# Autodesk Inventor assembly: B_Legs0
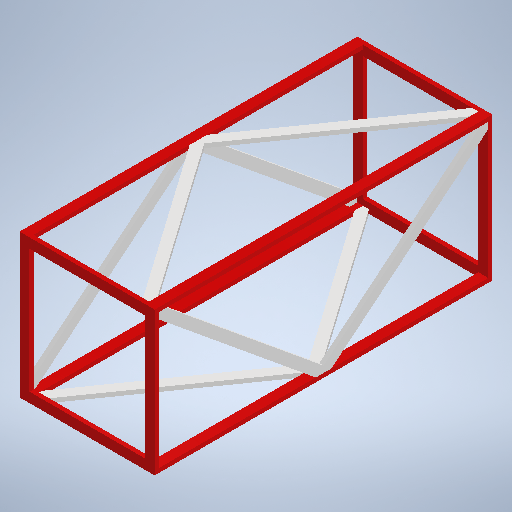
[picture p0: Inventor's stored thumbnail of the model, 512x512]
Saved by Autodesk Inventor 2025.1 (Build 291241020, 241B)
## iProperties
Created: 2024-09-19
Part Number: B_Legs0
Document SubType Name: Assembly
Designer: User
Author: User
## Documents named in this file (6)
- C:\Users\User\Documents\Tburn24\F_Legs1\B_Legs0.iam
- C:\Users\User\Documents\Tburn24\F_Legs1\8'x2x4.ipt
- C:\Users\User\Documents\Tburn24\F_Legs1\3'5x2x4.ipt
- C:\Users\User\Documents\Tburn24\F_Legs1\4x2x4.ipt
- C:\Users\User\Documents\Tburn24\F_Legs1\side1.ipt
- C:\Users\User\Documents\Tburn24\F_Legs1\side2.ipt
## Components (16 placed, 5 different names)
1. 8'x2x4:1 — Flush:1, Flush:2, Flush:3, Flush:8, Mate:3, Flush:10, Flush:12, Flush:13, Flush:14, Flush:22
2. 8'x2x4:2 — Mate:1, Flush:1, Flush:2, Flush:3, Mate:5, Flush:9, Flush:11, Flush:15, Flush:16, Flush:27, Mate:19, Flush:31, Mate:21, Flush:32
3. 4x2x4:1 — Flush:8, Flush:13, Flush:14, Mate:7, Flush:17, Flush:20, Mate:14, Mate:15, Flush:21, Mate:16, Flush:23, Flush:29
4. 4x2x4:2 — Mate:5, Flush:15, Flush:16, Mate:6, Flush:18, Flush:19, Mate:22
5. 4x2x4:3 — Flush:9, Flush:11, Flush:25, Flush:26
6. 4x2x4:4 — Mate:3, Flush:10, Flush:12, Mate:17, Mate:18
7. 8'x2x4:3 — Mate:7, Flush:17, Flush:20, Mate:14, Flush:24, Flush:30
8. 8'x2x4:4 — Mate:6, Flush:18, Flush:19, Flush:28
9. 3'5x2x4:1 — Mate:15, Flush:21, Flush:22
10. 3'5x2x4:2 — Mate:16, Flush:23, Flush:24
11. 3'5x2x4:3 — Mate:18, Flush:25, Flush:28
12. 3'5x2x4:4 — Mate:17, Flush:26, Flush:27, Mate:20
13. side1:1 — Flush:29
14. side2:1 — Flush:30
15. side2:2 — Mate:19, Mate:20, Flush:31
16. side1:2 — Mate:21, Mate:22, Flush:32
## Relationships (42: Flush 28, Mate 14)
- Mate:1: 8'x2x4:2
- Flush:1: 8'x2x4:1 ↔ 8'x2x4:2
- Flush:2 (1130.3 mm): 8'x2x4:1 ↔ 8'x2x4:2
- Flush:3: 8'x2x4:1 ↔ 8'x2x4:2
- Flush:8: 8'x2x4:1 ↔ 4x2x4:1
- Mate:3: 8'x2x4:1 ↔ 4x2x4:4
- Mate:5: 8'x2x4:2 ↔ 4x2x4:2
- Flush:9: 8'x2x4:2 ↔ 4x2x4:3
- Flush:10: 8'x2x4:1 ↔ 4x2x4:4
- Flush:11: 8'x2x4:2 ↔ 4x2x4:3
- Flush:12: 8'x2x4:1 ↔ 4x2x4:4
- Flush:13: 8'x2x4:1 ↔ 4x2x4:1
- Flush:14: 8'x2x4:1 ↔ 4x2x4:1
- Flush:15: 8'x2x4:2 ↔ 4x2x4:2
- Flush:16: 8'x2x4:2 ↔ 4x2x4:2
- Mate:6: 4x2x4:2 ↔ 8'x2x4:4
- Mate:7: 4x2x4:1 ↔ 8'x2x4:3
- Flush:17: 4x2x4:1 ↔ 8'x2x4:3
- Flush:18: 4x2x4:2 ↔ 8'x2x4:4
- Flush:19: 4x2x4:2 ↔ 8'x2x4:4
- Flush:20: 4x2x4:1 ↔ 8'x2x4:3
- Mate:14: 4x2x4:1 ↔ 8'x2x4:3
- Mate:15: 4x2x4:1 ↔ 3'5x2x4:1
- Flush:21: 4x2x4:1 ↔ 3'5x2x4:1
- Flush:22: 8'x2x4:1 ↔ 3'5x2x4:1
- Mate:16: 4x2x4:1 ↔ 3'5x2x4:2
- Flush:23: 4x2x4:1 ↔ 3'5x2x4:2
- Flush:24: 8'x2x4:3 ↔ 3'5x2x4:2
- Mate:17: 4x2x4:4 ↔ 3'5x2x4:4
- Mate:18: 4x2x4:4 ↔ 3'5x2x4:3
- Flush:25: 4x2x4:3 ↔ 3'5x2x4:3
- Flush:26: 4x2x4:3 ↔ 3'5x2x4:4
- Flush:27: 8'x2x4:2 ↔ 3'5x2x4:4
- Flush:28: 8'x2x4:4 ↔ 3'5x2x4:3
- Flush:29: 4x2x4:1 ↔ side1:1
- Flush:30: 8'x2x4:3 ↔ side2:1
- Mate:19: 8'x2x4:2 ↔ side2:2
- Mate:20: 3'5x2x4:4 ↔ side2:2
- Flush:31: 8'x2x4:2 ↔ side2:2
- Mate:21: 8'x2x4:2 ↔ side1:2
- Mate:22: 4x2x4:2 ↔ side1:2
- Flush:32: 8'x2x4:2 ↔ side1:2
